# Autodesk Inventor assembly: am-3637 NeveRest 20 Orbital Gearmotor
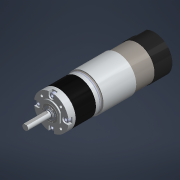
[picture p0: Inventor's stored thumbnail of the model, 180x180]
Saved by Autodesk Inventor 2022 (Build 260153000, 153)
## iProperties
Created: 2017-08-09
Part Number: am-3637 NeveRest 20 Orbital Gearmotor
Description: STEP AP214
Document SubType Name: Assembly
Designer: izack
Sending System: SolidWorks 2017
Preprocessor: SwSTEP 2.0
Title: am-3637 NeveRest 20 Orbital Gearmotor.STEP
Revision Number: ANY
## Documents named in this file (8)
- D:\Robotics\ComputerAidedDesign\2021-22\FTC\Parts\AndyMark\am-3637 NeveRest 20 Orbital Gearmotor.iam
- D:\Robotics\ComputerAidedDesign\2021-22\FTC\Parts\AndyMark\NeveRest orbital 2 stage Gearbox.ipt
- D:\Robotics\ComputerAidedDesign\2021-22\FTC\Parts\AndyMark\SHCS M3 x 16mm.ipt
- D:\Robotics\ComputerAidedDesign\2021-22\FTC\Parts\AndyMark\7804K117_STAINLESS STEEL BALL BEARING_7804K117.ipt
- D:\Robotics\ComputerAidedDesign\2021-22\FTC\Parts\AndyMark\97633A150_BLACK-FINISH STEEL EXTERNAL RETAINING RING_97633A150_grv.ipt
- D:\Robotics\ComputerAidedDesign\2021-22\FTC\Parts\AndyMark\Shim.ipt
- D:\Robotics\ComputerAidedDesign\2021-22\FTC\Parts\AndyMark\am-3104 NeveRest Motor.ipt
- D:\Robotics\ComputerAidedDesign\NeveRest 20 Orbiital Mount.ipt
## Components (10 placed, 10 different names)
1. NeveRest orbital 2 stage Gearbox_1 — Flush:1, Rigid:1
2. SHCS M3 x 16mm_2
3. SHCS M3 x 16mm_3
4. SHCS M3 x 16mm_4
5. SHCS M3 x 16mm_5
6. 7804K117_STAINLESS STEEL BALL BEARING_7804K117_6
7. 97633A150_BLACK-FINISH STEEL EXTERNAL RETAINING RING_97633A150_grv_7
8. Shim_8
9. am-3104 NeveRest Motor_9 — Rigid:1
10. NeveRest 20 Orbiital Mount:1 — Flush:1
## Relationships (2: Flush 1, WeldJoint 1)
- Flush:1: NeveRest orbital 2 stage Gearbox_1 ↔ NeveRest 20 Orbiital Mount:1
- Rigid:1 [WeldJoint]: NeveRest orbital 2 stage Gearbox_1 ↔ am-3104 NeveRest Motor_9
